# Autodesk Inventor assembly: testAssambly
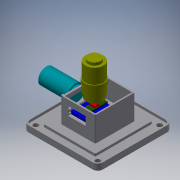
[picture p0: Inventor's stored thumbnail of the model, 180x180]
Saved by Autodesk Inventor 2016 (Build 200138000, 138)
## iProperties
Created: 2016-11-02
Part Number: testAssambly
Document SubType Name: Assembly
Designer: sims01
Author: sims01
## Documents named in this file (9)
- H:\Documents\LSFM_3\setup\mechanical\design\sampleHolderDesign\testAssambly.iam
- H:\Documents\LSFM_3\setup\mechanical\design\sampleHolderDesign\sampleChamberExt.ipt
- H:\Documents\LSFM_3\setup\mechanical\design\lsfm3_mechDesign\olympusXLSLPLN25XGMP_vFIN.ipt
- H:\Documents\LSFM_3\setup\mechanical\design\lsfm3_mechDesign\10X_mitutoyoObj.ipt
- H:\Documents\LSFM_3\setup\mechanical\design\sampleHolderDesign\sampleChamberInterior.ipt
- H:\Documents\LSFM_3\setup\mechanical\design\sampleHolderDesign\siliconBase.ipt
- H:\Documents\LSFM_3\setup\mechanical\design\sampleHolderDesign\filipeSample.ipt
- H:\Documents\LSFM_3\setup\mechanical\design\sampleHolderDesign\sampleHolderXYstageBase.ipt
- H:\Documents\LSFM_3\setup\mechanical\design\sampleHolderDesign\sampleChamber.ipt
## Components (8 placed, 8 different names)
1. sampleChamberExt:1
2. olympusXLSLPLN25XGMP_vFIN:1 — Mate:1, Mate:2, Mate:3, Rigid:4
3. 10X_mitutoyoObj:1 — Mate:4, Mate:5, Mate:6
4. sampleChamberInterior:1 — Flush:1, Rigid:2, Rigid:6
5. siliconBase:1 — Rigid:2, Rigid:3
6. filipeSample:1 — Rigid:3, Rigid:4
7. sampleHolderXYstageBase:1 — Rigid:5
8. sampleChamber:1 — Rigid:5, Rigid:6
## Relationships (12: Mate 6, WeldJoint 5, Flush 1)
- Mate:1: olympusXLSLPLN25XGMP_vFIN:1
- Mate:2 (8 mm): olympusXLSLPLN25XGMP_vFIN:1
- Mate:3: olympusXLSLPLN25XGMP_vFIN:1
- Mate:4: 10X_mitutoyoObj:1
- Mate:5: 10X_mitutoyoObj:1
- Mate:6 (-33 mm): 10X_mitutoyoObj:1
- Flush:1: sampleChamberInterior:1
- Rigid:2 [WeldJoint]: sampleChamberInterior:1 ↔ siliconBase:1
- Rigid:3 [WeldJoint]: siliconBase:1 ↔ filipeSample:1
- Rigid:4 [WeldJoint] (8 mm): olympusXLSLPLN25XGMP_vFIN:1 ↔ filipeSample:1
- Rigid:5 [WeldJoint]: sampleHolderXYstageBase:1 ↔ sampleChamber:1
- Rigid:6 [WeldJoint]: sampleChamberInterior:1 ↔ sampleChamber:1
